# Autodesk Inventor assembly: Assembly 2.0 upload
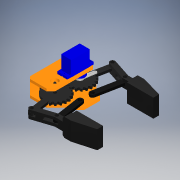
[picture p0: Inventor's stored thumbnail of the model, 180x180]
Saved by Autodesk Inventor 2021 (Build 250183000, 183)
## iProperties
Created: 2021-04-25
Part Number: Assembly 2.0 upload
Document SubType Name: Assembly
Designer: Luthfi
Author: Luthfi
## Documents named in this file (8)
- D:\Work\inventor\TA Arm Robot\gripper gear\Assembly 2.0 upload.iam
- D:\Work\inventor\TA Arm Robot\gripper gear\gear.ipt
- D:\Work\inventor\TA Arm Robot\gripper gear\gripper.ipt
- D:\Work\inventor\TA Arm Robot\gripper gear\lever.ipt
- D:\Work\inventor\TA Arm Robot\gripper gear\microservoSG90.ipt
- D:\Work\inventor\TA Arm Robot\gripper gear\gear 2.1.ipt
- D:\Work\inventor\TA Arm Robot\TA Kelompok 4 TME 3\sg90 servo\servo horn 1 v2.ipt
- D:\Work\inventor\TA Arm Robot\gripper gear\base 2.0 upload.ipt
## Components (9 placed, 7 different names)
1. gear:1 — Insert:5, Insert:18
2. gripper:1 — Insert:7, Insert:12
3. lever:1 — Insert:7, Insert:20
4. gripper:2 — Insert:5, Insert:8
5. lever:2 — Insert:8, Insert:21
6. microservoSG90:1 — Insert:17, Insert:22, Insert:23
7. gear 2.1:1 — Insert:12, Mate:1, Insert:19
8. servo horn 1 v2:1 — Insert:17, Mate:1
9. base 2.0 upload:1 — Insert:18, Insert:19, Insert:20, Insert:21, Insert:22, Insert:23
## Relationships (12: Insert 11, Mate 1)
- Insert:5: gear:1 ↔ gripper:2
- Insert:7: gripper:1 ↔ lever:1
- Insert:8: gripper:2 ↔ lever:2
- Insert:12: gripper:1 ↔ gear 2.1:1
- Insert:17: microservoSG90:1 ↔ servo horn 1 v2:1
- Mate:1: gear 2.1:1 ↔ servo horn 1 v2:1
- Insert:18: gear:1 ↔ base 2.0 upload:1
- Insert:19: gear 2.1:1 ↔ base 2.0 upload:1
- Insert:20: lever:1 ↔ base 2.0 upload:1
- Insert:21: lever:2 ↔ base 2.0 upload:1
- Insert:22: microservoSG90:1 ↔ base 2.0 upload:1
- Insert:23: microservoSG90:1 ↔ base 2.0 upload:1
